# Autodesk Inventor assembly: SecondWheelAssembl
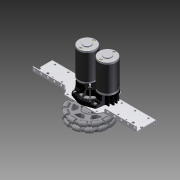
[picture p0: Inventor's stored thumbnail of the model, 180x180]
Saved by Autodesk Inventor 2015 (Build 190159000, 159)
## iProperties
Created: 2015-01-17
Part Number: SecondWheelAssembl
Document SubType Name: Assembly
Designer: jhirshland1
Author: jhirshland1
## Documents named in this file (3)
- C:\Users\jhirshland1\Inventor\HWRobot2015\FRCKOP2015\AndyMark\SecondWheelAssembl.iam
- C:\Users\jhirshland1\Inventor\HWRobot2015\FRCKOP2015\Drive Base\am-2952 AM14U2 Inside Sheet.ipt
- C:\Users\jhirshland1\Inventor\HWRobot2015\FRCKOP2015\AndyMark\WheelAssembly.iam
## Components (2 placed, 2 different names)
1. am-2952 AM14U2 Inside Sheet:1
2. WheelAssembly:1 [sub-assembly]
## Relationships (2: Insert 2)
- [Insert]: am-2952 AM14U2 Inside Sheet:1 ↔ WheelAssembly:1
- [Insert]: am-2952 AM14U2 Inside Sheet:1 ↔ WheelAssembly:1
## Named parameters: d105_d103 = 0 mm, d106_d104 = 0 mm
